# Autodesk Inventor assembly: RPLIDAR A1M8 kit(iges)
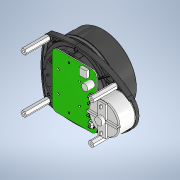
[picture p0: Inventor's stored thumbnail of the model, 180x180]
Saved by Autodesk Inventor 2020 (Build 240168000, 168)
## iProperties
Created: 2021-06-01
Part Number: RPLIDAR A1M8 kit(iges)
Description: SolidWorks IGES file using analytic representation for surfaces
Document SubType Name: Assembly
Designer: Антон
Sending System: SolidWorks 2020
Preprocessor: SolidWorks 2020
Minimum Resolution: 0.0
Sending System Product ID: ϞП-RPLIDAR-1.5 - R6
Receiving System Product ID: ϞП-RPLIDAR-1.5 - R6
Sent Units: Millimeter
Translation Standard: IGES 5.3
Model Creation Time: 2021-06-01
Author: WangYC
## Documents named in this file (23)
- D:\Project\Robots\Новая папка\FutureEngineersViolet\3D-models\RRO 2021 Mk. IV\Components\RPLIDAR A1M8\RPLIDAR A1M8.iam
- D:\Project\Robots\Новая папка\FutureEngineersViolet\3D-models\RRO 2021 Mk. IV\Components\RPLIDAR A1M8\6807.ipt
- D:\Project\Robots\Новая папка\FutureEngineersViolet\3D-models\RRO 2021 Mk. IV\Components\RPLIDAR A1M8\ϞПѽתƽ̨1.5.ipt
- D:\Project\Robots\Новая папка\FutureEngineersViolet\3D-models\RRO 2021 Mk. IV\Components\RPLIDAR A1M8\Ý׹2.ipt
- D:\Project\Robots\Новая папка\FutureEngineersViolet\3D-models\RRO 2021 Mk. IV\Components\RPLIDAR A1M8\1.25 4pin.ipt
- D:\Project\Robots\Новая папка\FutureEngineersViolet\3D-models\RRO 2021 Mk. IV\Components\RPLIDAR A1M8\1.25 3pinb͹.ipt
- D:\Project\Robots\Новая папка\FutureEngineersViolet\3D-models\RRO 2021 Mk. IV\Components\RPLIDAR A1M8\1.25 2pin-2.ipt
- D:\Project\Robots\Новая папка\FutureEngineersViolet\3D-models\RRO 2021 Mk. IV\Components\RPLIDAR A1M8\1.25 2pin-1.ipt
- D:\Project\Robots\Новая папка\FutureEngineersViolet\3D-models\RRO 2021 Mk. IV\Components\RPLIDAR A1M8\short metal version-2.ipt
- D:\Project\Robots\FutureEngineersViolet\3D-models\RRO 2021 Mk. IV\Components\RPLIDAR A1M8\ϞПힿ�ힿ�ƽ̨1.5.ipt
- D:\Project\Robots\Новая папка\FutureEngineersViolet\3D-models\RRO 2021 Mk. IV\Components\RPLIDAR A1M8\ힿ�˕PCBힿ�1.5.ipt
- D:\Project\Robots\Новая папка\FutureEngineersViolet\3D-models\RRO 2021 Mk. IV\Components\RPLIDAR A1M8\ힿ�ힿ�ힿ�вힿ�1.5.ipt
- D:\Project\Robots\Новая папка\FutureEngineersViolet\3D-models\RRO 2021 Mk. IV\Components\RPLIDAR A1M8\ힿ�ͷힿ�вힿ�1.5.ipt
- D:\Project\Robots\FutureEngineersViolet\3D-models\RRO 2021 Mk. IV\Components\RPLIDAR A1M8\Բ̨ힿ�1.5.ipt
- D:\Project\Robots\Новая папка\FutureEngineersViolet\3D-models\RRO 2021 Mk. IV\Components\RPLIDAR A1M8\ힿ�ힿ�.ipt
- D:\Project\Robots\Новая папка\FutureEngineersViolet\3D-models\RRO 2021 Mk. IV\Components\RPLIDAR A1M8\Ƥힿ�Ö1.5.ipt
- D:\Project\Robots\Новая папка\FutureEngineersViolet\3D-models\RRO 2021 Mk. IV\Components\RPLIDAR A1M8\ힿ�ͷ.ipt
- D:\Project\Robots\Новая папка\FutureEngineersViolet\3D-models\RRO 2021 Mk. IV\Components\RPLIDAR A1M8\ힿ�ëǷ.ipt
- D:\Project\Robots\Новая папка\FutureEngineersViolet\3D-models\RRO 2021 Mk. IV\Components\RPLIDAR A1M8\Ƥힿ�1-5^ϞП-RPLIDAR-1.5 - R6.ipt
- D:\Project\Robots\Новая папка\FutureEngineersViolet\3D-models\RRO 2021 Mk. IV\Components\RPLIDAR A1M8\ힿ�ʤPCB1.5V2.ipt
- D:\Project\Robots\FutureEngineersViolet\3D-models\RRO 2021 Mk. IV\Components\RPLIDAR A1M8\ͭힿ�Ȧ.ipt
- D:\Project\Robots\Новая папка\FutureEngineersViolet\3D-models\RRO 2021 Mk. IV\Components\RPLIDAR A1M8\ힿ�ힿ�Ƿ.ipt
- D:\Project\Robots\Новая папка\FutureEngineersViolet\3D-models\RRO 2021 Mk. IV\Components\RPLIDAR A1M8\ힿ�ힿ�1.7 -тힿ�ힿ�.ipt
## Components (12 placed, 9 different names)
1. 6807 — С поворотом:2, С поворотом:3
2. ϞПѽתƽ̨1.5 — Жесткий:7, Жесткий:8, Жесткий:9, Жесткий:16, С поворотом:2, С поворотом:21
3. Ƥힿ�Ö1.5 — С поворотом:1, С поворотом:22
4. short metal version-2 — Жесткий:10, Жесткий:11, Жесткий:12, Жесткий:13, Жесткий:14, Жесткий:15
5. 1.25 4pin
6. 1.25 3pinb͹
7. 1.25 2pin-2
8. 1.25 2pin-1
9. Ý׹2 — Жесткий:3
10. Ý׹2:1 — Жесткий:4
11. Ý׹2:2 — Жесткий:5
12. Ý׹2:3 — Жесткий:2
## Relationships (24: WeldJoint 17, RevoluteJoint 7)
- Жесткий:1 [WeldJoint]
- Жесткий:2 [WeldJoint]: Ý׹2:3
- Жесткий:3 [WeldJoint]: Ý׹2
- Жесткий:4 [WeldJoint]: Ý׹2:1
- Жесткий:5 [WeldJoint]: Ý׹2:2
- Жесткий:6 [WeldJoint]
- С поворотом:1 [RevoluteJoint]: Ƥힿ�Ö1.5
- Жесткий:7 [WeldJoint]: ϞПѽתƽ̨1.5
- Жесткий:8 [WeldJoint]: ϞПѽתƽ̨1.5
- Жесткий:9 [WeldJoint]: ϞПѽתƽ̨1.5
- Жесткий:10 [WeldJoint] (2 mm): short metal version-2
- Жесткий:11 [WeldJoint]: short metal version-2
- Жесткий:12 [WeldJoint]: short metal version-2
- Жесткий:13 [WeldJoint]: short metal version-2
- Жесткий:14 [WeldJoint]: short metal version-2
- Жесткий:15 [WeldJoint]: short metal version-2
- Жесткий:16 [WeldJoint]: ϞПѽתƽ̨1.5
- Жесткий:17 [WeldJoint] (0.5 mm)
- С поворотом:2 [RevoluteJoint]: 6807 ↔ ϞПѽתƽ̨1.5
- С поворотом:3 [RevoluteJoint]: 6807
- С поворотом:19 [RevoluteJoint]
- С поворотом:20 [RevoluteJoint]
- С поворотом:21 [RevoluteJoint]: ϞПѽתƽ̨1.5
- С поворотом:22 [RevoluteJoint]: Ƥힿ�Ö1.5
